# Autodesk Inventor assembly: Cockpit_back_frame
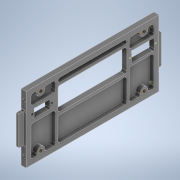
[picture p0: Inventor's stored thumbnail of the model, 180x180]
Saved by Autodesk Inventor 2022.3 (Build 263350000, 350)
## iProperties
Created: 2023-05-17
Part Number: Cockpit_back_frame
Document SubType Name: Assembly
Designer: Masato Kubotera
Author: Masato Kubotera
## Documents named in this file (4)
- C:\Users\Masato\Documents\Inventor\Inventor for CIT Brains\SUSTAINA-OP - Cockpit mate\UpperBody\Cockpit\Cockpit_back_frame.iam
- C:\Users\Masato\Documents\Inventor\Inventor for CIT Brains\SUSTAINA-OP - Cockpit mate\UpperBody\Cockpit\Cockpit_back_frame.ipt
- C:\Users\Masato\Documents\Inventor\Inventor for CIT Brains\SUSTAINA-OP - Cockpit mate\ReadyMade\InsertNut\IRU-304S.ipt
- C:\Users\Masato\Documents\Inventor\Inventor for CIT Brains\SUSTAINA-OP - Cockpit mate\ReadyMade\InsertNut\UD-43040.ipt
## Components (9 placed, 3 different names)
1. Cockpit_back_frame:1 — フラッシュ:1, フラッシュ:2, フラッシュ:3, 挿入:1, 挿入:2, 挿入:3, 挿入:4, 挿入:5, 挿入:6, 挿入:7, 挿入:8
2. IRU-304S:1 — 挿入:1
3. UD-43040:1 — 挿入:5
4. IRU-304S:2 — 挿入:2
5. UD-43040:2 — 挿入:6
6. IRU-304S:3 — 挿入:3
7. UD-43040:3 — 挿入:7
8. IRU-304S:4 — 挿入:4
9. UD-43040:4 — 挿入:8
## Relationships (11: Insert 8, Flush 3)
- フラッシュ:1 [Flush]: Cockpit_back_frame:1
- フラッシュ:2 [Flush]: Cockpit_back_frame:1
- フラッシュ:3 [Flush]: Cockpit_back_frame:1
- 挿入:1 [Insert]: Cockpit_back_frame:1 ↔ IRU-304S:1
- 挿入:2 [Insert]: Cockpit_back_frame:1 ↔ IRU-304S:2
- 挿入:3 [Insert]: Cockpit_back_frame:1 ↔ IRU-304S:3
- 挿入:4 [Insert]: Cockpit_back_frame:1 ↔ IRU-304S:4
- 挿入:5 [Insert]: Cockpit_back_frame:1 ↔ UD-43040:1
- 挿入:6 [Insert]: Cockpit_back_frame:1 ↔ UD-43040:2
- 挿入:7 [Insert]: Cockpit_back_frame:1 ↔ UD-43040:3
- 挿入:8 [Insert]: Cockpit_back_frame:1 ↔ UD-43040:4
